# Autodesk Inventor assembly: Assembly1
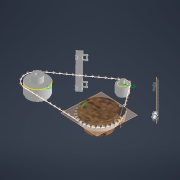
[picture p0: Inventor's stored thumbnail of the model, 180x180]
Saved by Autodesk Inventor 2022 (Build 260153000, 153)
## iProperties
Created: 2021-12-29
Part Number: Assembly1
Document SubType Name: Assembly
Designer: MatusBarany
Author: MatusBarany
## Documents named in this file (9)
- C:\Users\Public\Documents\Autodesk\Inventor 2022\Projects\wall-e\Assembly1.iam
- C:\Users\Public\Documents\Autodesk\Inventor 2022\Projects\wall-e\chain ink.ipt
- C:\Users\Public\Documents\Autodesk\Inventor 2022\Projects\wall-e\chain ink_outer.ipt
- C:\Users\Public\Documents\Autodesk\Inventor 2022\Projects\wall-e\male_koliesko.ipt
- C:\Users\Public\Documents\Autodesk\Inventor 2022\Projects\wall-e\velke_koleso.ipt
- C:\Users\Public\Documents\Autodesk\Inventor 2022\Projects\wall-e\stredne_koleso.ipt
- C:\Users\Public\Documents\Autodesk\Inventor 2022\Projects\wall-e\path of chain.ipt
- C:\Users\Public\Documents\Autodesk\Inventor 2022\Projects\wall-e\onePart_chain.ipt
- C:\Users\Public\Documents\Autodesk\Inventor 2022\Projects\chain_test\Link - High Strength Chain.ipt
## Components (9 placed, 8 different names)
1. chain ink:1 — Cylindrical:1, Cylindrical:4
2. chain ink_outer:1 — Cylindrical:1
3. chain ink_outer:2 — Cylindrical:4
4. male_koliesko:1
5. velke_koleso:1 — Flush:1
6. stredne_koleso:1
7. path of chain:1 — Mate:1, Mate:2
8. onePart_chain:1
9. Link - High Strength Chain:1 — Flush:2, Mate:1, Mate:2
## Relationships (6: CylindricalJoint 2, Flush 2, Mate 2)
- Cylindrical:1: chain ink:1 ↔ chain ink_outer:1
- Cylindrical:4: chain ink:1 ↔ chain ink_outer:2
- Flush:1 (-1.5 mm): velke_koleso:1
- Flush:2: Link - High Strength Chain:1
- Mate:1: path of chain:1 ↔ Link - High Strength Chain:1
- Mate:2: path of chain:1 ↔ Link - High Strength Chain:1
